# Autodesk Inventor assembly: Montagem2
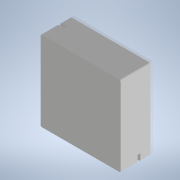
[picture p0: Inventor's stored thumbnail of the model, 180x180]
Saved by Autodesk Inventor 2022 (Build 260153000, 153)
## iProperties
Created: 2022-03-13
Part Number: Montagem2
Document SubType Name: Assembly
Designer: Hanter
Author: Hanter
## Documents named in this file (7)
- G:\Meu Drive\Projetos\Projeto 2020 2021\Eletrônica 2020-2021\Projeção mecânica\caixa transmissao\Montagem2.iam
- G:\Meu Drive\Projetos\Projeto 2020 2021\Eletrônica 2020-2021\Projeção mecânica\caixa transmissao\caixa transmissao.ipt
- G:\Meu Drive\Projetos\Projeto 2020 2021\Eletrônica 2020-2021\Projeção mecânica\caixa transmissao\tampa hc12.ipt
- G:\Meu Drive\Projetos\Projeto 2020 2021\Eletrônica 2020-2021\Projeção mecânica\caixa transmissao\Placa Trasmissao.ipt
- G:\Meu Drive\Projetos\Projeto 2020 2021\Eletrônica 2020-2021\Projeção mecânica\caixa transmissao\Regulador.ipt
- G:\Meu Drive\Projetos\Projeto 2020 2021\Eletrônica 2020-2021\Projeção mecânica\caixa transmissao\tampa caixa.ipt
- G:\Meu Drive\Projetos\Projeto 2020 2021\Eletrônica 2020-2021\Projeção mecânica\caixa transmissao\AMP 3 position.ipt
## Components (8 placed, 6 different names)
1. caixa transmissao:1 — Coincidente:1, Coincidente:4, Coincidente:5, Coincidente:6, Coincidente:7, Coincidente:8, Coincidente:9, Coincidente:10, Coincidente:11, Coincidente:12, Coincidente:13, Coincidente:14, Coincidente:15, Coincidente:16
2. tampa hc12:1 — Coincidente:1
3. Placa Trasmissao:1 — Coincidente:7, Coincidente:8, Coincidente:9
4. Regulador:1 — Coincidente:4, Coincidente:5, Coincidente:6
5. tampa caixa:1 — Coincidente:10
6. AMP 3 position:1 — Coincidente:11, Coincidente:12
7. AMP 3 position:2 — Coincidente:13, Coincidente:14
8. AMP 3 position:3 — Coincidente:15, Coincidente:16
## Relationships (14: Mate 14)
- Coincidente:1 [Mate]: caixa transmissao:1 ↔ tampa hc12:1
- Coincidente:4 [Mate]: caixa transmissao:1 ↔ Regulador:1
- Coincidente:5 [Mate]: caixa transmissao:1 ↔ Regulador:1
- Coincidente:6 [Mate]: caixa transmissao:1 ↔ Regulador:1
- Coincidente:7 [Mate]: caixa transmissao:1 ↔ Placa Trasmissao:1
- Coincidente:8 [Mate]: caixa transmissao:1 ↔ Placa Trasmissao:1
- Coincidente:9 [Mate]: caixa transmissao:1 ↔ Placa Trasmissao:1
- Coincidente:10 [Mate]: caixa transmissao:1 ↔ tampa caixa:1
- Coincidente:11 [Mate]: caixa transmissao:1 ↔ AMP 3 position:1
- Coincidente:12 [Mate]: caixa transmissao:1 ↔ AMP 3 position:1
- Coincidente:13 [Mate]: caixa transmissao:1 ↔ AMP 3 position:2
- Coincidente:14 [Mate]: caixa transmissao:1 ↔ AMP 3 position:2
- Coincidente:15 [Mate]: caixa transmissao:1 ↔ AMP 3 position:3
- Coincidente:16 [Mate]: caixa transmissao:1 ↔ AMP 3 position:3
